# Autodesk Inventor assembly: Rail_Animation
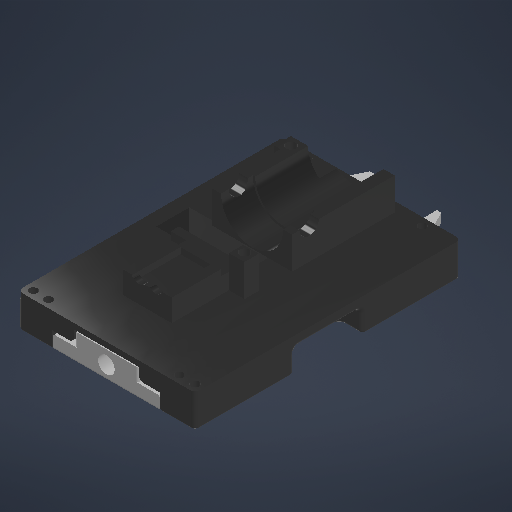
[picture p0: Inventor's stored thumbnail of the model, 512x512]
Saved by Autodesk Inventor 2026.2 (Build 302298000, 298)
## iProperties
Created: 2026-03-31
Part Number: Rail_Animation
Document SubType Name: Assembly
Designer: vckot
Author: vckot
## Documents named in this file (4)
- C:\Users\vckot\OneDrive\Documents\Vaibhav\capstone\CAD_files\Version_6\Rail_Animation.iam
- C:\Users\vckot\OneDrive\Documents\Vaibhav\capstone\CAD_files\Version_6\PCB_Housing_01_V4.ipt
- C:\Users\vckot\OneDrive\Documents\Vaibhav\capstone\CAD_files\Version_6\Tourniquet_Rail_01_V4.ipt
- C:\Users\vckot\OneDrive\Documents\Vaibhav\capstone\CAD_files\Version_6\Tubing_Male_Connector.ipt
## Components (3 placed, 3 different names)
1. PCB_Housing_01_V4:1 — Flush:1, Flush:2, Flush:3, Flush:4, Mate:3, Flush:5
2. Tourniquet_Rail_01_V4:1 — Mate:1, Mate:2, Flush:4, Mate:3, Flush:5
3. Tubing_Male_Connector:1 — Mate:1, Mate:2
## Relationships (8: Flush 5, Mate 3)
- Flush:1: PCB_Housing_01_V4:1
- Flush:2: PCB_Housing_01_V4:1
- Flush:3: PCB_Housing_01_V4:1
- Mate:1: Tourniquet_Rail_01_V4:1 ↔ Tubing_Male_Connector:1
- Mate:2 (12 mm): Tourniquet_Rail_01_V4:1 ↔ Tubing_Male_Connector:1
- Flush:4: PCB_Housing_01_V4:1 ↔ Tourniquet_Rail_01_V4:1
- Mate:3: PCB_Housing_01_V4:1 ↔ Tourniquet_Rail_01_V4:1
- Flush:5: PCB_Housing_01_V4:1 ↔ Tourniquet_Rail_01_V4:1
